# Autodesk Inventor assembly: Flotador
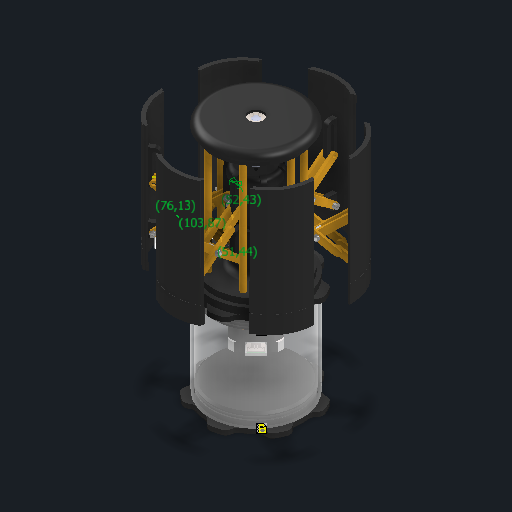
[picture p0: Inventor's stored thumbnail of the model, 512x512]
Saved by Autodesk Inventor 2025.3 (Build 293356030, 356C)
## iProperties
Created: 2024-12-25
Part Number: Flotador
Document SubType Name: Assembly
Designer: Usuario
Mass: 2248.45 g
Surface Area: 3887.08 cm^2
Volume: 903.403 cm^3
Density: 2.48886 g/cm^3
Author: Usuario
## Documents named in this file (5)
- C:\Users\santa\OneDrive - Universidad de los Andes\Robocol\Flotador\V3\Flotador.iam
- C:\Users\santa\OneDrive - Universidad de los Andes\Robocol\Flotador\V3\Chasis.iam
- C:\Users\santa\OneDrive - Universidad de los Andes\Robocol\Flotador\V3\Expansor.iam
- C:\Users\santa\OneDrive - Universidad de los Andes\Robocol\Flotador\Downloads\17HS4401S Stepper Motor\17HS4401S Stepper Motor_SUB.ipt
- C:\Users\santa\OneDrive - Universidad de los Andes\Robocol\Flotador\Downloads\lead screw 8mm\lead screw 8mm.ipt
## Components (4 placed, 4 different names)
1. Chasis:1 [sub-assembly] — Nivelación:1, Nivelación:2, Nivelación:3, Rígido:1, Rígido:2
2. Expansor:1 [sub-assembly] — Rígido:1, Coincidencia:1
3. 17HS4401S Stepper Motor_SUB:1 — Rígido:2
4. lead screw 8mm:1
## Relationships (6: Flush 3, WeldJoint 2, Mate 1)
- Nivelación:1 [Flush]: Chasis:1
- Nivelación:2 [Flush]: Chasis:1
- Nivelación:3 [Flush]: Chasis:1
- Rígido:1 [WeldJoint]: Chasis:1 ↔ Expansor:1
- Rígido:2 [WeldJoint]: Chasis:1 ↔ 17HS4401S Stepper Motor_SUB:1
- Coincidencia:1 [Mate]: Expansor:1
